# Autodesk Inventor assembly: Piston_Housing
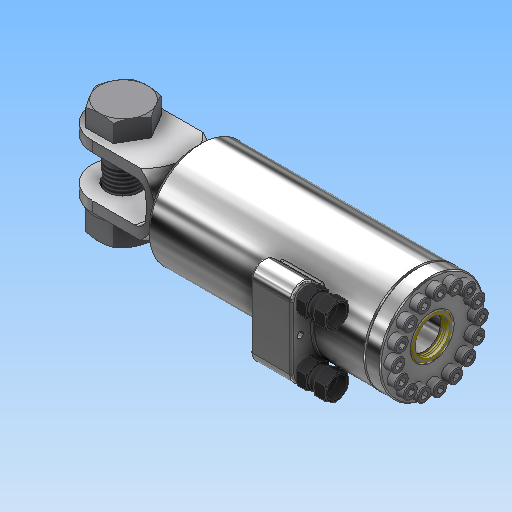
[picture p0: Inventor's stored thumbnail of the model, 512x512]
Saved by Autodesk Inventor 2020.1 (Build 241239000, 239)
## iProperties
Created: 2003-05-03
Part Number: Piston_Housing
Document SubType Name: Assembly
Designer: Stephen Hooper
Manufacturer: Standard
Standards Organization: Custom
Control State: 0
Master: False
Checked Out: False
Shininess: 64.0
Length Units: 11269
Angle Units: 11279
Time Units: 11290
Mass Units: 11283
Length Display Precision: 3
Angle Display Precision: 2
Compacted: True
Density: 0.0
Volumn: 0.0
Area: 0.0
PropertySet Name: Model Information
Author: Stephen Hooper
## Documents named in this file (11)
- C:\Users\thomastremblay\Desktop\Inventor ACP Data\Assemblies\Piston_Housing.iam
- C:\Users\thomastremblay\Desktop\Inventor ACP Data\Parts\Piston_Housing.ipt
- C:\Users\thomastremblay\Desktop\Inventor ACP Data\Parts\Cylinder_Cap.ipt
- C:\Users\thomastremblay\Desktop\Inventor ACP Data\Content Center\3176 Fitting.ipt
- C:\Users\thomastremblay\Desktop\Inventor ACP Data\Parts\Housing_Connector.ipt
- C:\Users\thomastremblay\Desktop\Inventor ACP Data\Parts\Collar_Seal_Inner.ipt
- C:\Users\thomastremblay\Desktop\Inventor ACP Data\Parts\Collar_Seal_Outer.ipt
- C:\Users\thomastremblay\Desktop\Inventor ACP Data\Content Center\local.BSI.12.750.5.ipt
- C:\Users\thomastremblay\Desktop\Inventor ACP Data\Content Center\local.BSI.47.140.5.ipt
- C:\Users\thomastremblay\Desktop\Inventor ACP Data\Content Center\local.BSI.30.190.5.ipt
- C:\Users\thomastremblay\Desktop\Inventor ACP Data\Content Center\local.BSI.6.3030.5.ipt
## Components (26 placed, 10 different names)
1. Piston_Housing:1 — Mate:1, Mate:2, Angle:1, Mate:6, Mate:7, Angle:2, Insert:5, Insert:6
2. Cylinder_Cap:1 — Mate:3, Mate:4, Flush:1, Mate:5, Insert:1, Mate:6, Mate:7, Angle:2
3. Housing_Connector:1 — Mate:1, Mate:2, Angle:1, Insert:2, Insert:3
4. Collar_Seal_Inner:1 — Mate:3, Mate:4
5. Collar_Seal_Outer:1 — Flush:1, Mate:5
6. BS 3692  Hexagon Head Screw  (Regular Thread - Metric) M30 x 90:2 — Insert:2
7. BS 4320  Form E M30 (Form E):2 — Insert:3, Insert:4
8. BS 3692  (Regular Thread - Metric) M30:2 — Insert:4
9. 3176 Fitting:1 — Insert:5
10. 3176 Fitting:2 — Insert:6
11. BS 4168 : Part 1  Hexagon Socket Head Cap Screw  (Regular Thread - Metric) M8 x 35:1 — Insert:1
12. BS 4168 : Part 1  Hexagon Socket Head Cap Screw  (Regular Thread - Metric) M8 x 35:16
13. BS 4168 : Part 1  Hexagon Socket Head Cap Screw  (Regular Thread - Metric) M8 x 35:17
14. BS 4168 : Part 1  Hexagon Socket Head Cap Screw  (Regular Thread - Metric) M8 x 35:18
15. BS 4168 : Part 1  Hexagon Socket Head Cap Screw  (Regular Thread - Metric) M8 x 35:19
16. BS 4168 : Part 1  Hexagon Socket Head Cap Screw  (Regular Thread - Metric) M8 x 35:20
17. BS 4168 : Part 1  Hexagon Socket Head Cap Screw  (Regular Thread - Metric) M8 x 35:21
18. BS 4168 : Part 1  Hexagon Socket Head Cap Screw  (Regular Thread - Metric) M8 x 35:22
19. BS 4168 : Part 1  Hexagon Socket Head Cap Screw  (Regular Thread - Metric) M8 x 35:23
20. BS 4168 : Part 1  Hexagon Socket Head Cap Screw  (Regular Thread - Metric) M8 x 35:24
21. BS 4168 : Part 1  Hexagon Socket Head Cap Screw  (Regular Thread - Metric) M8 x 35:25
22. BS 4168 : Part 1  Hexagon Socket Head Cap Screw  (Regular Thread - Metric) M8 x 35:26
23. BS 4168 : Part 1  Hexagon Socket Head Cap Screw  (Regular Thread - Metric) M8 x 35:27
24. BS 4168 : Part 1  Hexagon Socket Head Cap Screw  (Regular Thread - Metric) M8 x 35:28
25. BS 4168 : Part 1  Hexagon Socket Head Cap Screw  (Regular Thread - Metric) M8 x 35:29
26. BS 4168 : Part 1  Hexagon Socket Head Cap Screw  (Regular Thread - Metric) M8 x 35:30
## Component patterns: (16 elements, first: BS 4168 : Part 1  Hexagon Socket Head Cap Screw  (Regular Thread - Metric) M8 x 35:1)
## Relationships (16: Mate 7, Insert 6, Angle 2, Flush 1)
- Mate:1: Piston_Housing:1 ↔ Housing_Connector:1
- Mate:2: Piston_Housing:1 ↔ Housing_Connector:1
- Angle:1 (0 deg): Piston_Housing:1 ↔ Housing_Connector:1
- Mate:3: Cylinder_Cap:1 ↔ Collar_Seal_Inner:1
- Mate:4: Cylinder_Cap:1 ↔ Collar_Seal_Inner:1
- Flush:1: Cylinder_Cap:1 ↔ Collar_Seal_Outer:1
- Mate:5: Cylinder_Cap:1 ↔ Collar_Seal_Outer:1
- Insert:1: Cylinder_Cap:1 ↔ BS 4168 : Part 1  Hexagon Socket Head Cap Screw  (Regular Thread - Metric) M8 x 35:1
- Insert:2: Housing_Connector:1 ↔ BS 3692  Hexagon Head Screw  (Regular Thread - Metric) M30 x 90:2
- Insert:3: Housing_Connector:1 ↔ BS 4320  Form E M30 (Form E):2
- Insert:4: BS 4320  Form E M30 (Form E):2 ↔ BS 3692  (Regular Thread - Metric) M30:2
- Mate:6: Piston_Housing:1 ↔ Cylinder_Cap:1
- Mate:7: Piston_Housing:1 ↔ Cylinder_Cap:1
- Angle:2 (0 deg): Piston_Housing:1 ↔ Cylinder_Cap:1
- Insert:5: Piston_Housing:1 ↔ 3176 Fitting:1
- Insert:6: Piston_Housing:1 ↔ 3176 Fitting:2
